# Autodesk Inventor assembly: Assembly1
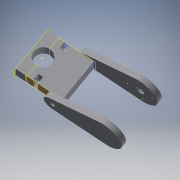
[picture p0: Inventor's stored thumbnail of the model, 180x180]
Saved by Autodesk Inventor 2018 (Build 220112000, 112)
## iProperties
Created: 2017-06-05
Part Number: Assembly1
Document SubType Name: Assembly
Designer: Zadeka
Author: Zadeka
## Documents named in this file (5)
- C:\Users\Zadeka\Desktop\New folder\Assembly1.iam
- C:\Users\Zadeka\Desktop\New folder\BIKE.ipt
- C:\Users\Zadeka\Desktop\New folder\motormount.ipt
- C:\Users\Zadeka\Desktop\New folder\Part2.ipt
- C:\Users\Zadeka\Desktop\New folder\mounpt2.ipt
## Components (4 placed, 4 different names)
1. BIKE:1 — Rotational:1, Rotational:2, Rotational:3, Rotational:4
2. motormount:1 — Rotational:2, Mate:1
3. Part2:1 — Rotational:1, Mate:1
4. mounpt2:1 — Rotational:3, Rotational:4
## Relationships (5: RevoluteJoint 4, Mate 1)
- Rotational:1 [RevoluteJoint]: BIKE:1 ↔ Part2:1
- Rotational:2 [RevoluteJoint]: BIKE:1 ↔ motormount:1
- Mate:1: motormount:1 ↔ Part2:1
- Rotational:3 [RevoluteJoint]: BIKE:1 ↔ mounpt2:1
- Rotational:4 [RevoluteJoint]: BIKE:1 ↔ mounpt2:1
